# Autodesk Inventor assembly: 1x1
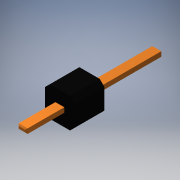
[picture p0: Inventor's stored thumbnail of the model, 180x180]
Saved by Autodesk Inventor 2016 (Build 200138000, 138)
## iProperties
Created: 2014-07-19
Part Number: 1x1
Document SubType Name: Assembly
Designer: Sawaiz Syed
Author: Sawaiz Syed
## Documents named in this file (3)
- C:\Users\Jonathan\Documents\Projects\dynodePiShield\coincidenceCounter\cad\electronics\2.54 breakaway\1x1.iam
- C:\Users\Jonathan\Documents\Projects\dynodePiShield\coincidenceCounter\cad\electronics\2.54 breakaway\Holder.ipt
- C:\Users\Jonathan\Documents\Projects\dynodePiShield\coincidenceCounter\cad\electronics\2.54 breakaway\Pin.ipt
## Components (2 placed, 2 different names)
1. Holder:1 — Mate:1, Mate:2, Flush:1
2. Pin:1 — Mate:1, Mate:2, Flush:1
## Relationships (3: Mate 2, Flush 1)
- Mate:1: Holder:1 ↔ Pin:1
- Mate:2: Holder:1 ↔ Pin:1
- Flush:1 (-5.84 mm): Holder:1 ↔ Pin:1
